# Autodesk Inventor assembly: robocik
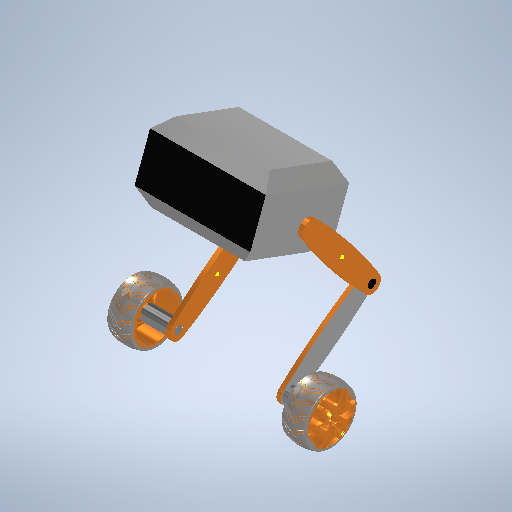
[picture p0: Inventor's stored thumbnail of the model, 512x512]
Saved by Autodesk Inventor 2025 (Build 290162000, 162)
## iProperties
Created: 2024-04-21
Part Number: robocik
Document SubType Name: Assembly
Designer: joann
Author: joann
## Documents named in this file (8)
- C:\Users\joann\Desktop\Inventor\RM\robocik.iam
- C:\Users\joann\Desktop\Inventor\RM\silniczek.ipt
- C:\Users\joann\Desktop\Inventor\RM\silniczek_MIR.ipt
- C:\Users\joann\Desktop\Inventor\RM\odnoga1.ipt
- C:\Users\joann\Desktop\Inventor\RM\tire.ipt
- C:\Users\joann\Desktop\Inventor\RM\rim.ipt
- C:\Users\joann\Desktop\Inventor\RM\rim_MIR.ipt
- C:\Users\joann\Desktop\Inventor\RM\bloczek.ipt
## Components (11 placed, 7 different names)
1. silniczek_MIR:1 — Mate:1, Insert:2, Insert:8
2. silniczek:1 — Mate:1, Insert:1, Insert:7
3. odnoga1:2 — Insert:1, Insert:3
4. odnoga1:3 — Insert:3, Insert:10
5. odnoga1:4 — Insert:4, Insert:9
6. odnoga1:5 — Insert:2, Insert:4
7. tire:1 — Insert:6
8. tire:2 — Insert:5
9. rim:2 — Insert:6, Insert:7
10. rim_MIR:1 — Insert:5, Insert:8
11. bloczek:1 — Insert:9, Insert:10
## Relationships (11: Insert 10, Mate 1)
- Mate:1: silniczek_MIR:1 ↔ silniczek:1
- Insert:1: silniczek:1 ↔ odnoga1:2
- Insert:2: silniczek_MIR:1 ↔ odnoga1:5
- Insert:3: odnoga1:2 ↔ odnoga1:3
- Insert:4: odnoga1:4 ↔ odnoga1:5
- Insert:5: tire:2 ↔ rim_MIR:1
- Insert:6: tire:1 ↔ rim:2
- Insert:7: silniczek:1 ↔ rim:2
- Insert:8: silniczek_MIR:1 ↔ rim_MIR:1
- Insert:9: odnoga1:4 ↔ bloczek:1
- Insert:10: odnoga1:3 ↔ bloczek:1
